# Autodesk Inventor assembly: Baugruppe3
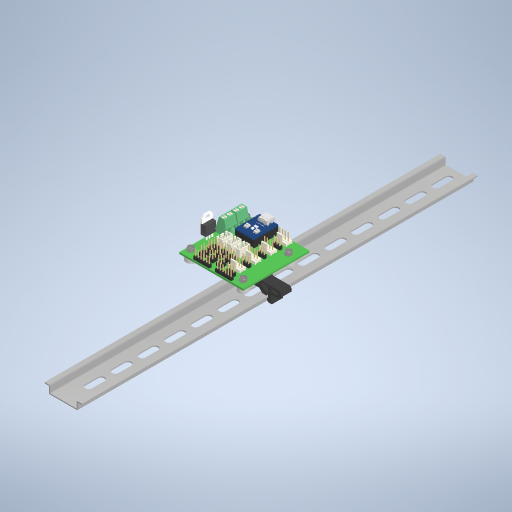
[picture p0: Inventor's stored thumbnail of the model, 512x512]
Saved by Autodesk Inventor 2023.1 (Build 271208000, 208)
## iProperties
Created: 2022-09-15
Part Number: Baugruppe3
Document SubType Name: Assembly
Designer: Rama
Author: Rama
## Documents named in this file (7)
- C:\Users\Rama\Desktop\TinyFan\CAD\SRC\TinyFan_Dinrail_Assembled.iam
- C:\Users\Rama\Desktop\TinyFan\CAD\SRC\TinyFan_DinRail.ipt
- C:\Users\Rama\Desktop\GitHub\Voron-2-Mods\DinClips\CAD\SRC\New_DinClip_Insert.ipt
- C:\Users\Rama\Desktop\GitHub\TrashInventor\M3 Threaded Insert.ipt
- C:\Users\Rama\Documents\Inventor\Content Center Files\R2023\de-DE\DIN 912\DIN 912 - M3 x 0,5 x 8 x 6,75.ipt
- C:\Users\Rama\Desktop\TinyFan\CAD\SRC\TinyFan_V2.iam
- C:\Users\Rama\Desktop\GitHub\TrashInventor\DIN3 Rail.ipt
## Components (16 placed, 6 different names)
1. TinyFan_DinRail:1 — Passend:2, Passend:3, Passend:6, Passend:7, Passend:8, Passend:9, Passend:10, Passend:11, Passend:12, Passend:13, Passend:18, Fluchtend:9, Passend:20, Passend:21
2. New_DinClip_Insert:1 — Passend:2, Passend:3, Passend:4, Passend:5, Fluchtend:10, Passend:20, Passend:22, Passend:23
3. M3 Threaded Insert:1 — Passend:4, Fluchtend:1, Fluchtend:10
4. M3 Threaded Insert:2 — Passend:5, Fluchtend:1
5. M3 Threaded Insert:3 — Passend:6, Fluchtend:2
6. M3 Threaded Insert:4 — Passend:9, Fluchtend:2, Fluchtend:3
7. M3 Threaded Insert:5 — Passend:7, Fluchtend:3, Fluchtend:4
8. M3 Threaded Insert:6 — Passend:8, Fluchtend:4, Fluchtend:9
9. DIN 912 - ersetzt durch DIN EN ISO 4762 M3 x 8:1 — Passend:11, Fluchtend:5
10. DIN 912 - ersetzt durch DIN EN ISO 4762 M3 x 8:2 — Passend:10, Fluchtend:5, Passend:18
11. TinyFan_V2:1 [sub-assembly] — Passend:12, Passend:13, Passend:14, Passend:15, Passend:16, Passend:17, Passend:19, Passend:21
12. DIN 912 - ersetzt durch DIN EN ISO 4762 M3 x 8:3 — Passend:14, Fluchtend:8
13. DIN 912 - ersetzt durch DIN EN ISO 4762 M3 x 8:4 — Passend:17, Fluchtend:6
14. DIN 912 - ersetzt durch DIN EN ISO 4762 M3 x 8:5 — Passend:16, Fluchtend:6, Fluchtend:7, Passend:19
15. DIN 912 - ersetzt durch DIN EN ISO 4762 M3 x 8:6 — Passend:15, Fluchtend:7, Fluchtend:8
16. DIN3 Rail:1 — Passend:22, Passend:23
## Relationships (32: Mate 22, Flush 10)
- Passend:2 [Mate]: TinyFan_DinRail:1 ↔ New_DinClip_Insert:1
- Passend:3 [Mate]: TinyFan_DinRail:1 ↔ New_DinClip_Insert:1
- Passend:4 [Mate]: New_DinClip_Insert:1 ↔ M3 Threaded Insert:1
- Passend:5 [Mate]: New_DinClip_Insert:1 ↔ M3 Threaded Insert:2
- Fluchtend:1 [Flush]: M3 Threaded Insert:1 ↔ M3 Threaded Insert:2
- Passend:6 [Mate]: TinyFan_DinRail:1 ↔ M3 Threaded Insert:3
- Passend:7 [Mate]: TinyFan_DinRail:1 ↔ M3 Threaded Insert:5
- Passend:8 [Mate]: TinyFan_DinRail:1 ↔ M3 Threaded Insert:6
- Passend:9 [Mate]: TinyFan_DinRail:1 ↔ M3 Threaded Insert:4
- Fluchtend:2 [Flush]: M3 Threaded Insert:3 ↔ M3 Threaded Insert:4
- Fluchtend:3 [Flush]: M3 Threaded Insert:4 ↔ M3 Threaded Insert:5
- Fluchtend:4 [Flush]: M3 Threaded Insert:5 ↔ M3 Threaded Insert:6
- Passend:10 [Mate]: TinyFan_DinRail:1 ↔ DIN 912 - ersetzt durch DIN EN ISO 4762 M3 x 8:2
- Passend:11 [Mate]: TinyFan_DinRail:1 ↔ DIN 912 - ersetzt durch DIN EN ISO 4762 M3 x 8:1
- Fluchtend:5 [Flush]: DIN 912 - ersetzt durch DIN EN ISO 4762 M3 x 8:1 ↔ DIN 912 - ersetzt durch DIN EN ISO 4762 M3 x 8:2
- Passend:12 [Mate]: TinyFan_DinRail:1 ↔ TinyFan_V2:1
- Passend:13 [Mate]: TinyFan_DinRail:1 ↔ TinyFan_V2:1
- Passend:14 [Mate]: TinyFan_V2:1 ↔ DIN 912 - ersetzt durch DIN EN ISO 4762 M3 x 8:3
- Passend:15 [Mate]: TinyFan_V2:1 ↔ DIN 912 - ersetzt durch DIN EN ISO 4762 M3 x 8:6
- Passend:16 [Mate]: TinyFan_V2:1 ↔ DIN 912 - ersetzt durch DIN EN ISO 4762 M3 x 8:5
- Passend:17 [Mate]: TinyFan_V2:1 ↔ DIN 912 - ersetzt durch DIN EN ISO 4762 M3 x 8:4
- Fluchtend:6 [Flush]: DIN 912 - ersetzt durch DIN EN ISO 4762 M3 x 8:4 ↔ DIN 912 - ersetzt durch DIN EN ISO 4762 M3 x 8:5
- Fluchtend:7 [Flush]: DIN 912 - ersetzt durch DIN EN ISO 4762 M3 x 8:5 ↔ DIN 912 - ersetzt durch DIN EN ISO 4762 M3 x 8:6
- Fluchtend:8 [Flush]: DIN 912 - ersetzt durch DIN EN ISO 4762 M3 x 8:3 ↔ DIN 912 - ersetzt durch DIN EN ISO 4762 M3 x 8:6
- Passend:18 [Mate]: TinyFan_DinRail:1 ↔ DIN 912 - ersetzt durch DIN EN ISO 4762 M3 x 8:2
- Passend:19 [Mate]: TinyFan_V2:1 ↔ DIN 912 - ersetzt durch DIN EN ISO 4762 M3 x 8:5
- Fluchtend:9 [Flush]: TinyFan_DinRail:1 ↔ M3 Threaded Insert:6
- Fluchtend:10 [Flush]: New_DinClip_Insert:1 ↔ M3 Threaded Insert:1
- Passend:20 [Mate]: TinyFan_DinRail:1 ↔ New_DinClip_Insert:1
- Passend:21 [Mate]: TinyFan_DinRail:1 ↔ TinyFan_V2:1
- Passend:22 [Mate]: New_DinClip_Insert:1 ↔ DIN3 Rail:1
- Passend:23 [Mate]: New_DinClip_Insert:1 ↔ DIN3 Rail:1
